# Autodesk Inventor assembly: Clamp with Piston Assembly
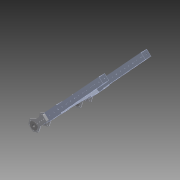
[picture p0: Inventor's stored thumbnail of the model, 180x180]
Saved by Autodesk Inventor 2014 SP1 (Build 180222100, 222)
## iProperties
Created: 2014-01-12
Part Number: Clamp with Piston Assembly
Document SubType Name: Assembly
Designer: Michael
Mass: 537.07 g
Surface Area: 2462.83 cm^2
Volume: 181.546 cm^3
Density: 2.95832 g/cm^3
Author: Michael
## Documents named in this file (7)
- C:\Users\Arpan\Documents\GitHub\2014buildCAD\New Collector\Clamp with Piston Assembly.iam
- C:\Users\Arpan\Documents\GitHub\2014buildCAD\New Collector\Vex Pro 1x1 rectangular tubing 14 in length.ipt
- C:\Users\Arpan\Documents\GitHub\2014buildCAD\Duluth Collector\Bearing Mount Spacer 1-8 in.ipt
- C:\Users\Arpan\Documents\GitHub\2014buildCAD\New Collector\Vex Pro 1x1 rectangular tubing 6 in length.ipt
- C:\Users\Arpan\Documents\GitHub\2014buildCAD\New Collector\Hex Bearing 3-8 in (FR6ZZL-hex (am-0692)).ipt
- C:\Users\Arpan\Documents\GitHub\2014buildCAD\New Collector\Vex Pro End Bearing Mount (Bolt).ipt
- C:\Users\Arpan\Documents\GitHub\2014buildCAD\New Collector\Vex Pro Versa Chassis Gusset.ipt
## Components (19 placed, 6 different names)
1. Vex Pro 1x1 rectangular tubing 14 in length:1 — Mate:184, Mate:185, Mate:186, Mate:189, Mate:190, Mate:191, Flush:1, Mate:207, Mate:208, Mate:209, Mate:210, Mate:212, Mate:213
2. Vex Pro 1x1 rectangular tubing 14 in length:2 — Mate:193, Mate:194, Mate:195, Mate:197, Mate:198, Mate:199, Flush:1, Mate:206, Mate:214, Mate:215, Mate:216, Mate:217, Mate:218, Mate:219
3. Bearing Mount Spacer 1-8 in:1 — Mate:171, Mate:172, Mate:173, Mate:207, Mate:208
4. Bearing Mount Spacer 1-8 in:2 — Mate:166, Mate:167, Mate:168, Mate:210, Mate:213
5. Vex Pro 1x1 rectangular tubing 6 in length:2 — Mate:187, Mate:188, Mate:192, Mate:196, Mate:200, Mate:205
6. Bearing Mount Spacer 1-8 in:7 — Mate:176, Mate:177, Mate:178, Mate:214
7. Bearing Mount Spacer 1-8 in:9 — Mate:181, Mate:182, Mate:183, Mate:206, Mate:217, Mate:218, Mate:219
8. Hex Bearing 3-8 in (FR6ZZL-hex (am-0692)):1 — Mate:174, Mate:175
9. Hex Bearing 3-8 in (FR6ZZL-hex (am-0692)):2 — Mate:201, Mate:202
10. Hex Bearing 3-8 in (FR6ZZL-hex (am-0692)):3 — Mate:203, Mate:204
11. Hex Bearing 3-8 in (FR6ZZL-hex (am-0692)):4 — Mate:179, Mate:180
12. Vex Pro End Bearing Mount (Bolt):1 — Mate:166, Mate:167, Mate:168, Mate:201, Mate:202, Mate:212
13. Vex Pro End Bearing Mount (Bolt):2 — Mate:171, Mate:172, Mate:173, Mate:174, Mate:175, Mate:209
14. Vex Pro End Bearing Mount (Bolt):3 — Mate:176, Mate:177, Mate:178, Mate:179, Mate:180, Mate:215, Mate:216
15. Vex Pro End Bearing Mount (Bolt):4 — Mate:181, Mate:182, Mate:183, Mate:203, Mate:204
16. Vex Pro Versa Chassis Gusset:1 — Mate:184, Mate:185, Mate:186, Mate:187, Mate:188
17. Vex Pro Versa Chassis Gusset:2 — Mate:189, Mate:190, Mate:191, Mate:192
18. Vex Pro Versa Chassis Gusset:3 — Mate:193, Mate:194, Mate:195, Mate:196
19. Vex Pro Versa Chassis Gusset:4 — Mate:197, Mate:198, Mate:199, Mate:200, Mate:205
## Relationships (52: Mate 51, Flush 1)
- Mate:166: Bearing Mount Spacer 1-8 in:2 ↔ Vex Pro End Bearing Mount (Bolt):1
- Mate:167: Bearing Mount Spacer 1-8 in:2 ↔ Vex Pro End Bearing Mount (Bolt):1
- Mate:168: Bearing Mount Spacer 1-8 in:2 ↔ Vex Pro End Bearing Mount (Bolt):1
- Mate:171: Bearing Mount Spacer 1-8 in:1 ↔ Vex Pro End Bearing Mount (Bolt):2
- Mate:172: Bearing Mount Spacer 1-8 in:1 ↔ Vex Pro End Bearing Mount (Bolt):2
- Mate:173: Bearing Mount Spacer 1-8 in:1 ↔ Vex Pro End Bearing Mount (Bolt):2
- Mate:174: Hex Bearing 3-8 in (FR6ZZL-hex (am-0692)):1 ↔ Vex Pro End Bearing Mount (Bolt):2
- Mate:175: Hex Bearing 3-8 in (FR6ZZL-hex (am-0692)):1 ↔ Vex Pro End Bearing Mount (Bolt):2
- Mate:176: Bearing Mount Spacer 1-8 in:7 ↔ Vex Pro End Bearing Mount (Bolt):3
- Mate:177: Bearing Mount Spacer 1-8 in:7 ↔ Vex Pro End Bearing Mount (Bolt):3
- Mate:178: Bearing Mount Spacer 1-8 in:7 ↔ Vex Pro End Bearing Mount (Bolt):3
- Mate:179: Hex Bearing 3-8 in (FR6ZZL-hex (am-0692)):4 ↔ Vex Pro End Bearing Mount (Bolt):3
- Mate:180: Hex Bearing 3-8 in (FR6ZZL-hex (am-0692)):4 ↔ Vex Pro End Bearing Mount (Bolt):3
- Mate:181: Bearing Mount Spacer 1-8 in:9 ↔ Vex Pro End Bearing Mount (Bolt):4
- Mate:182: Bearing Mount Spacer 1-8 in:9 ↔ Vex Pro End Bearing Mount (Bolt):4
- Mate:183: Bearing Mount Spacer 1-8 in:9 ↔ Vex Pro End Bearing Mount (Bolt):4
- Mate:184: Vex Pro 1x1 rectangular tubing 14 in length:1 ↔ Vex Pro Versa Chassis Gusset:1
- Mate:185: Vex Pro 1x1 rectangular tubing 14 in length:1 ↔ Vex Pro Versa Chassis Gusset:1
- Mate:186: Vex Pro 1x1 rectangular tubing 14 in length:1 ↔ Vex Pro Versa Chassis Gusset:1
- Mate:187: Vex Pro 1x1 rectangular tubing 6 in length:2 ↔ Vex Pro Versa Chassis Gusset:1
- Mate:188: Vex Pro 1x1 rectangular tubing 6 in length:2 ↔ Vex Pro Versa Chassis Gusset:1
- Mate:189: Vex Pro 1x1 rectangular tubing 14 in length:1 ↔ Vex Pro Versa Chassis Gusset:2
- Mate:190: Vex Pro 1x1 rectangular tubing 14 in length:1 ↔ Vex Pro Versa Chassis Gusset:2
- Mate:191: Vex Pro 1x1 rectangular tubing 14 in length:1 ↔ Vex Pro Versa Chassis Gusset:2
- Mate:192: Vex Pro 1x1 rectangular tubing 6 in length:2 ↔ Vex Pro Versa Chassis Gusset:2
- Mate:193: Vex Pro 1x1 rectangular tubing 14 in length:2 ↔ Vex Pro Versa Chassis Gusset:3
- Mate:194: Vex Pro 1x1 rectangular tubing 14 in length:2 ↔ Vex Pro Versa Chassis Gusset:3
- Mate:195: Vex Pro 1x1 rectangular tubing 14 in length:2 ↔ Vex Pro Versa Chassis Gusset:3
- Mate:196: Vex Pro 1x1 rectangular tubing 6 in length:2 ↔ Vex Pro Versa Chassis Gusset:3
- Mate:197: Vex Pro 1x1 rectangular tubing 14 in length:2 ↔ Vex Pro Versa Chassis Gusset:4
- Mate:198: Vex Pro 1x1 rectangular tubing 14 in length:2 ↔ Vex Pro Versa Chassis Gusset:4
- Mate:199: Vex Pro 1x1 rectangular tubing 14 in length:2 ↔ Vex Pro Versa Chassis Gusset:4
- Mate:200: Vex Pro 1x1 rectangular tubing 6 in length:2 ↔ Vex Pro Versa Chassis Gusset:4
- Flush:1: Vex Pro 1x1 rectangular tubing 14 in length:1 ↔ Vex Pro 1x1 rectangular tubing 14 in length:2
- Mate:201: Hex Bearing 3-8 in (FR6ZZL-hex (am-0692)):2 ↔ Vex Pro End Bearing Mount (Bolt):1
- Mate:202: Hex Bearing 3-8 in (FR6ZZL-hex (am-0692)):2 ↔ Vex Pro End Bearing Mount (Bolt):1
- Mate:203: Hex Bearing 3-8 in (FR6ZZL-hex (am-0692)):3 ↔ Vex Pro End Bearing Mount (Bolt):4
- Mate:204: Hex Bearing 3-8 in (FR6ZZL-hex (am-0692)):3 ↔ Vex Pro End Bearing Mount (Bolt):4
- Mate:205: Vex Pro 1x1 rectangular tubing 6 in length:2 ↔ Vex Pro Versa Chassis Gusset:4
- Mate:206: Vex Pro 1x1 rectangular tubing 14 in length:2 ↔ Bearing Mount Spacer 1-8 in:9
- Mate:207: Vex Pro 1x1 rectangular tubing 14 in length:1 ↔ Bearing Mount Spacer 1-8 in:1
- Mate:208: Vex Pro 1x1 rectangular tubing 14 in length:1 ↔ Bearing Mount Spacer 1-8 in:1
- Mate:209: Vex Pro 1x1 rectangular tubing 14 in length:1 ↔ Vex Pro End Bearing Mount (Bolt):2
- Mate:210: Vex Pro 1x1 rectangular tubing 14 in length:1 ↔ Bearing Mount Spacer 1-8 in:2
- Mate:212: Vex Pro 1x1 rectangular tubing 14 in length:1 ↔ Vex Pro End Bearing Mount (Bolt):1
- Mate:213: Vex Pro 1x1 rectangular tubing 14 in length:1 ↔ Bearing Mount Spacer 1-8 in:2
- Mate:214: Vex Pro 1x1 rectangular tubing 14 in length:2 ↔ Bearing Mount Spacer 1-8 in:7
- Mate:215: Vex Pro 1x1 rectangular tubing 14 in length:2 ↔ Vex Pro End Bearing Mount (Bolt):3
- Mate:216: Vex Pro 1x1 rectangular tubing 14 in length:2 ↔ Vex Pro End Bearing Mount (Bolt):3
- Mate:217: Vex Pro 1x1 rectangular tubing 14 in length:2 ↔ Bearing Mount Spacer 1-8 in:9
- Mate:218: Vex Pro 1x1 rectangular tubing 14 in length:2 ↔ Bearing Mount Spacer 1-8 in:9
- Mate:219: Vex Pro 1x1 rectangular tubing 14 in length:2 ↔ Bearing Mount Spacer 1-8 in:9
